# Autodesk Inventor assembly: リンク_6_1
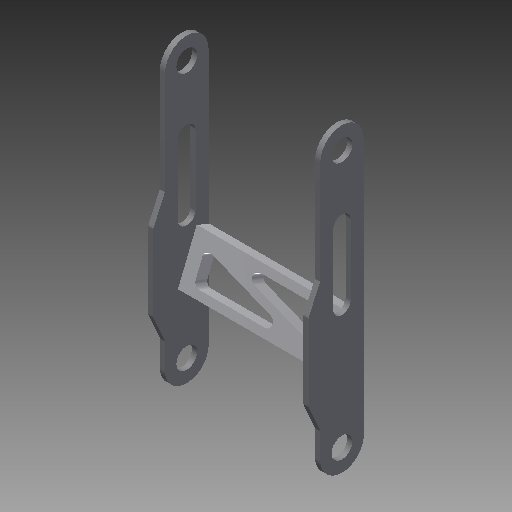
[picture p0: Inventor's stored thumbnail of the model, 512x512]
Saved by Autodesk Inventor 2018 (Build 220112000, 112)
## iProperties
Created: 2016-08-23
Part Number: リンク_6_1
Material: 一般
Document SubType Name: Assembly
Designer: hiro
Mass: 25.4181 g
Surface Area: 148.711 cm^2
Volume: 11.4997 cm^3
Density: 2.21034 g/cm^3
Author: hiro
## Documents named in this file (3)
- C:\Users\taka\Desktop\OPR\OpenPlatform_ver1_0\下半身_160823\リンク\リンク_6_1.iam
- C:\Users\taka\Desktop\OPR\OpenPlatform_ver1_0\下半身_160823\リンク\リンク_メインフレーム_6_3.ipt
- C:\Users\taka\Desktop\OPR\OpenPlatform_ver1_0\下半身_160823\リンク\リンク_サブフレーム_6_1.ipt
## Components (3 placed, 2 different names)
1. リンク_メインフレーム_6_3:1 — 挿入:30, 挿入:31, 挿入:32
2. リンク_メインフレーム_6_3:2 — 挿入:33, 挿入:34, 挿入:35
3. リンク_サブフレーム_6_1:1 — 挿入:30, 挿入:31, 挿入:32, 挿入:33, 挿入:34, 挿入:35
## Relationships (6: Insert 6)
- 挿入:30 [Insert]: リンク_メインフレーム_6_3:1 ↔ リンク_サブフレーム_6_1:1
- 挿入:31 [Insert]: リンク_メインフレーム_6_3:1 ↔ リンク_サブフレーム_6_1:1
- 挿入:32 [Insert]: リンク_メインフレーム_6_3:1 ↔ リンク_サブフレーム_6_1:1
- 挿入:33 [Insert]: リンク_メインフレーム_6_3:2 ↔ リンク_サブフレーム_6_1:1
- 挿入:34 [Insert]: リンク_メインフレーム_6_3:2 ↔ リンク_サブフレーム_6_1:1
- 挿入:35 [Insert]: リンク_メインフレーム_6_3:2 ↔ リンク_サブフレーム_6_1:1
